# Autodesk Inventor assembly: Assembly_XYTable_Aliepexress_cellstorm_laserslide
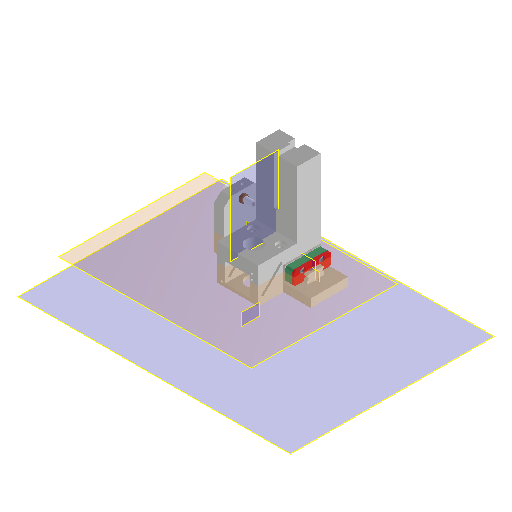
[picture p0: Inventor's stored thumbnail of the model, 512x512]
Saved by Autodesk Inventor 2022 (Build 260153000, 153)
## iProperties
Created: 2022-01-02
Part Number: Assembly_XYTable_Aliepexress_cellstorm_laserslide
Document SubType Name: Assembly
Designer: diederichbenedict
Author: diederichbenedict
## Documents named in this file (7)
- C:\Users\diederichbenedict\Dropbox\Dokumente\Promotion\PROJECTS\TIRFImager\INVENTOR\Assembly_XYTable_Aliepexress_cellstorm_laserslide.iam
- C:\Users\diederichbenedict\Dropbox\Dokumente\Promotion\PROJECTS\TIRFImager\INVENTOR\30_Cube_Z_Focus_MGN_NEMA_rail.ipt
- C:\Users\diederichbenedict\Dropbox\Dokumente\Promotion\PROJECTS\TIRFImager\INVENTOR\00_MGN12H, LINEAR GUIDE BLOCK.ipt
- C:\Users\diederichbenedict\Dropbox\Dokumente\Promotion\PROJECTS\TIRFImager\INVENTOR\30_XYTabel_Aliexpress_cellSTORM_xmount.ipt
- C:\Users\diederichbenedict\Dropbox\Dokumente\Promotion\PROJECTS\TIRFImager\INVENTOR\30_XYTabel_Aliexpress_cellSTORM_lasermount.ipt
- C:\Users\diederichbenedict\Dropbox\Dokumente\Promotion\PROJECTS\TIRFImager\INVENTOR\00_F6SSN2P-Step.ipt
- C:\Users\diederichbenedict\Dropbox\Dokumente\Promotion\PROJECTS\TIRFImager\INVENTOR\00_F6SS088-Step.ipt
## Components (6 placed, 6 different names)
1. 30_Cube_Z_Focus_MGN_NEMA_rail:1
2. 00_MGN12H, LINEAR GUIDE BLOCK:1
3. 30_XYTabel_Aliexpress_cellSTORM_xmount:1 — Einfügen:1
4. 30_XYTabel_Aliexpress_cellSTORM_lasermount:1
5. 00_F6SSN2P-Step:1 — Einfügen:1, Einfügen:2
6. 00_F6SS088-Step:1 — Einfügen:2
## Relationships (5: Mate 2, Insert 2, Flush 1)
- [Mate]: 30_Cube_Z_Focus_MGN_NEMA_rail:1 ↔ 00_MGN12H, LINEAR GUIDE BLOCK:1
- [Mate] (0.2 mm): 30_Cube_Z_Focus_MGN_NEMA_rail:1 ↔ 00_MGN12H, LINEAR GUIDE BLOCK:1
- [Flush]: 00_MGN12H, LINEAR GUIDE BLOCK:1 ↔ 30_XYTabel_Aliexpress_cellSTORM_lasermount:1
- Einfügen:1 [Insert]: 30_XYTabel_Aliexpress_cellSTORM_xmount:1 ↔ 00_F6SSN2P-Step:1
- Einfügen:2 [Insert] (-5 mm): 00_F6SSN2P-Step:1 ↔ 00_F6SS088-Step:1
